# Autodesk Inventor assembly: 117
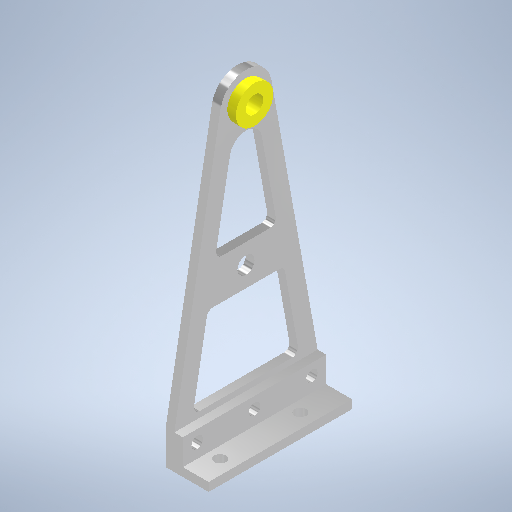
[picture p0: Inventor's stored thumbnail of the model, 512x512]
Saved by Autodesk Inventor 2025.1 (Build 291241000, 241)
## iProperties
Created: 2024-06-11
Part Number: 117
Document SubType Name: Assembly
Designer: ffogue
Author: ffogue
## Documents named in this file (4)
- C:\Users\ffogue\Downloads\Meine Projket\Paddle\117.iam
- C:\Users\ffogue\Downloads\Meine Projket\Paddle\1171.ipt
- C:\Users\ffogue\Downloads\Meine Projket\Paddle\1172.ipt
- C:\Users\ffogue\Downloads\Meine Projket\Paddle\1173.ipt
## Components (3 placed, 3 different names)
1. 1171:1 — Insert:1, Insert:2
2. 1172:1 — Insert:1
3. 1173:1 — Insert:2
## Relationships (2: Insert 2)
- Insert:1: 1171:1 ↔ 1172:1
- Insert:2: 1171:1 ↔ 1173:1
